# Autodesk Inventor assembly: Assembly_Cube_Laser_Block_v3
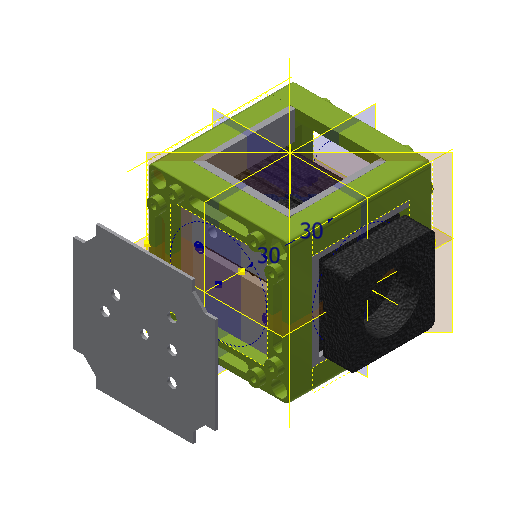
[picture p0: Inventor's stored thumbnail of the model, 512x512]
Saved by Autodesk Inventor 2022 (Build 260153000, 153)
## iProperties
Created: 2019-07-23
Part Number: Assembly_Cube_Laser_Block_v3
Document SubType Name: Assembly
Designer: marsikovabarbora
Mass: 41.9543 g
Surface Area: 260.494 cm^2
Volume: 37.9382 cm^3
Density: 1.10586 g/cm^3
Author: marsikovabarbora
## Documents named in this file (5)
- C:\Users\diederichbenedict\Dropbox\Dokumente\Promotion\PROJECTS\UC2-Hi2\INVENTOR\Assembly_Cube_Laser_Block_v3.iam
- C:\Users\diederichbenedict\Dropbox\Dokumente\Promotion\PROJECTS\UC2-Hi2\INVENTOR\Assembly_Cube_empty_IM_v3.iam
- C:\Users\diederichbenedict\Dropbox\Dokumente\Promotion\PROJECTS\UC2-Hi2\INVENTOR\00_Laser_532nm_200mw.ipt
- C:\Users\diederichbenedict\Dropbox\Dokumente\Promotion\PROJECTS\UC2-Hi2\INVENTOR\20_Cube_insert_AlliedVision_Alvium_v3.ipt
- C:\Users\diederichbenedict\Dropbox\Dokumente\Promotion\PROJECTS\UC2-Hi2\INVENTOR\20_Cube_insert_Laser_Block_adjustable_v3.ipt
## Components (4 placed, 4 different names)
1. Assembly_Cube_empty_IM_v3:1 [sub-assembly] — Mate:8, Angle:2, Flush:1, Flush:2, Flush:3
2. 00_Laser_532nm_200mw:1 — Mate:8, Angle:2, Flush:1
3. 20_Cube_insert_AlliedVision_Alvium_v3:1 — Flush:2, Flush:3
4. 20_Cube_insert_Laser_Block_adjustable_v3:2
## Relationships (9: Mate 5, Flush 3, Angle 1)
- [Mate]: Assembly_Cube_empty_IM_v3:1
- [Mate]: Assembly_Cube_empty_IM_v3:1
- [Mate]: Assembly_Cube_empty_IM_v3:1
- [Mate]: Assembly_Cube_empty_IM_v3:1 ↔ 00_Laser_532nm_200mw:1
- Mate:8: Assembly_Cube_empty_IM_v3:1 ↔ 00_Laser_532nm_200mw:1
- Angle:2 (0 deg): Assembly_Cube_empty_IM_v3:1 ↔ 00_Laser_532nm_200mw:1
- Flush:1: Assembly_Cube_empty_IM_v3:1 ↔ 00_Laser_532nm_200mw:1
- Flush:2 (-0.05 mm): Assembly_Cube_empty_IM_v3:1 ↔ 20_Cube_insert_AlliedVision_Alvium_v3:1
- Flush:3 (-0.05 mm): Assembly_Cube_empty_IM_v3:1 ↔ 20_Cube_insert_AlliedVision_Alvium_v3:1
